# Autodesk Inventor assembly: kolowahacz
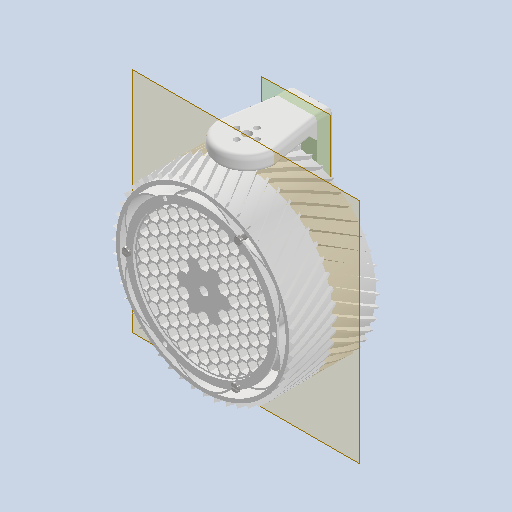
[picture p0: Inventor's stored thumbnail of the model, 512x512]
Saved by Autodesk Inventor 2025.3 (Build 293356000, 356)
## iProperties
Created: 2026-04-05
Part Number: kolowahacz
Document SubType Name: Assembly
Designer: ksawe
Author: ksawe
## Documents named in this file (3)
- C:\Users\ksawe\OneDrive\Pulpit\Exomy v1\wersja2\kolowahacz.iam
- C:\Users\ksawe\OneDrive\Pulpit\Exomy v1\wersja2\wahaczserwovol2.iam
- C:\Users\ksawe\OneDrive\Pulpit\Exomy v1\wersja2\kolo.iam
## Components (2 placed, 2 different names)
1. wahaczserwovol2:1 [sub-assembly] — Insert:1, Flush:2
2. kolo:1 [sub-assembly] — Insert:1, Flush:1
## Relationships (3: Flush 2, Insert 1)
- Insert:1: wahaczserwovol2:1 ↔ kolo:1
- Flush:1 (-30 mm): kolo:1
- Flush:2 (-12 mm): wahaczserwovol2:1
